# Autodesk Inventor assembly: WheelMountStack
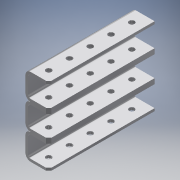
[picture p0: Inventor's stored thumbnail of the model, 180x180]
Saved by Autodesk Inventor 2016 (Build 200138000, 138)
## iProperties
Created: 2016-01-13
Part Number: WheelMountStack
Document SubType Name: Assembly
Designer: Administrator
Author: Administrator
## Documents named in this file (2)
- C:\Users\Administrator\Desktop\3192CAD\InitialRobotProto\WheelMountStack.iam
- C:\Users\Administrator\Desktop\3192CAD\InitialRobotProto\DBK_C-Channel_Tiny.ipt
## Components (3 placed, 1 different names)
1. DBK_C-Channel_Tiny:1 — Mate:1, Mate:2, Mate:3, Mate:4, Mate:5, Mate:6
2. DBK_C-Channel_Tiny:2 — Mate:1, Mate:4, Mate:6
3. DBK_C-Channel_Tiny:3 — Mate:2, Mate:3, Mate:5
## Relationships (6: Mate 6)
- Mate:1: DBK_C-Channel_Tiny:1 ↔ DBK_C-Channel_Tiny:2
- Mate:2: DBK_C-Channel_Tiny:1 ↔ DBK_C-Channel_Tiny:3
- Mate:3: DBK_C-Channel_Tiny:1 ↔ DBK_C-Channel_Tiny:3
- Mate:4: DBK_C-Channel_Tiny:1 ↔ DBK_C-Channel_Tiny:2
- Mate:5: DBK_C-Channel_Tiny:1 ↔ DBK_C-Channel_Tiny:3
- Mate:6: DBK_C-Channel_Tiny:1 ↔ DBK_C-Channel_Tiny:2
